# Autodesk Inventor assembly: EPS
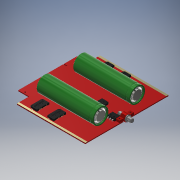
[picture p0: Inventor's stored thumbnail of the model, 180x180]
Saved by Autodesk Inventor 2018 (Build 220112000, 112)
## iProperties
Created: 2018-05-29
Part Number: EPS
Document SubType Name: Assembly
Designer: Bradley
Author: Bradley
## Documents named in this file (10)
- D:\Users\Bradley\Documents\CougsInSpace\CougSat1-Hardware\CougSat1-PowerBoard\CADModel\Native\EPS.iam
- D:\Users\Bradley\Documents\CougsInSpace\CougSat1-Hardware\CougSat1-PowerBoard\CADModel\Native\EPS_PCB.ipt
- D:\Users\Bradley\Documents\CougsInSpace\Resources\ComponentModels\Hardware\Pin_RBF.ipt
- D:\Users\Bradley\Documents\CougsInSpace\Resources\ComponentModels\Electronics\Switch_Micro-L.iam
- D:\Users\Bradley\Documents\CougsInSpace\Resources\ComponentModels\Electronics\Battery_18650.ipt
- D:\Users\Bradley\Documents\CougsInSpace\Resources\ComponentModels\Connectors\PicoLock--J-7.ipt
- D:\Users\Bradley\Documents\CougsInSpace\Resources\ComponentModels\Connectors\PicoLock--J-4.ipt
- D:\Users\Bradley\Documents\CougsInSpace\Resources\ComponentModels\Connectors\PicoLock--P-4.ipt
- D:\Users\Bradley\Documents\CougsInSpace\Resources\ComponentModels\Connectors\PicoLock--P-7.ipt
- D:\Users\Bradley\Documents\CougsInSpace\CougSat1-Hardware\CougSat1-PowerBoard\CADModel\Native\EPS_RBFPinHolder.ipt
## Components (16 placed, 9 different names)
1. EPS_PCB:1 — Mate:1, Angle:1, Flush:1, Flush:2, Mate:14, Mate:15, Mate:16, Mate:17, Mate:18, Flush:10, Flush:11, Flush:12, Flush:13, Flush:16, Mate:19, Insert:1, Insert:2
2. Pin_RBF:1 — Tangent:1, Insert:3
3. Switch_Micro-L:1 [sub-assembly] — Mate:1, Angle:1, Tangent:1, Mate:19
4. Battery_18650:1 — Flush:1, Flush:4, Symmetry:1
5. Battery_18650:2 — Flush:2, Flush:3, Symmetry:1
6. PicoLock--J-7:1 — Flush:6, Mate:6, Mate:7, Mate:14, Flush:10, Flush:14
7. PicoLock--J-4:1 — Flush:5, Mate:4, Mate:5, Mate:18
8. PicoLock--P-4:1 — Flush:5, Mate:4, Mate:5, Flush:16
9. PicoLock--P-7:1 — Flush:6, Mate:6, Mate:7
10. PicoLock--J-7:2 — Mate:15, Flush:11, Flush:15
11. PicoLock--P-7:2
12. PicoLock--J-7:3 — Mate:16, Flush:13, Flush:14
13. PicoLock--P-7:3
14. PicoLock--J-7:4 — Mate:17, Flush:12, Flush:15
15. PicoLock--P-7:4
16. EPS_RBFPinHolder:1 — Insert:1, Insert:2, Insert:3
## Relationships (39: Mate 17, Flush 16, Insert 3, Angle 1, Tangent 1, Symmetry 1)
- Mate:1: EPS_PCB:1 ↔ Switch_Micro-L:1
- Angle:1 (0 deg): EPS_PCB:1 ↔ Switch_Micro-L:1
- Tangent:1 (7.15 mm): Pin_RBF:1 ↔ Switch_Micro-L:1
- Flush:1 (-9 mm): EPS_PCB:1 ↔ Battery_18650:1
- Flush:2 (-9 mm): EPS_PCB:1 ↔ Battery_18650:2
- Flush:3 (-50 mm): Battery_18650:2
- Flush:4 (-50 mm): Battery_18650:1
- Symmetry:1: Battery_18650:1 ↔ Battery_18650:2
- Flush:5: PicoLock--J-4:1 ↔ PicoLock--P-4:1
- Mate:4: PicoLock--J-4:1 ↔ PicoLock--P-4:1
- Mate:5 (0.025 mm): PicoLock--J-4:1 ↔ PicoLock--P-4:1
- Flush:6: PicoLock--J-7:1 ↔ PicoLock--P-7:1
- Mate:6: PicoLock--J-7:1 ↔ PicoLock--P-7:1
- Mate:7 (0.025 mm): PicoLock--J-7:1 ↔ PicoLock--P-7:1
- [Flush]: PicoLock--J-7:2 ↔ PicoLock--P-7:2
- [Mate]: PicoLock--J-7:2 ↔ PicoLock--P-7:2
- [Mate] (0.025 mm): PicoLock--J-7:2 ↔ PicoLock--P-7:2
- [Flush]: PicoLock--J-7:3 ↔ PicoLock--P-7:3
- [Mate]: PicoLock--J-7:3 ↔ PicoLock--P-7:3
- [Mate] (0.025 mm): PicoLock--J-7:3 ↔ PicoLock--P-7:3
- [Flush]: PicoLock--J-7:4 ↔ PicoLock--P-7:4
- [Mate]: PicoLock--J-7:4 ↔ PicoLock--P-7:4
- [Mate] (0.025 mm): PicoLock--J-7:4 ↔ PicoLock--P-7:4
- Mate:14: EPS_PCB:1 ↔ PicoLock--J-7:1
- Mate:15: EPS_PCB:1 ↔ PicoLock--J-7:2
- Mate:16: EPS_PCB:1 ↔ PicoLock--J-7:3
- Mate:17: EPS_PCB:1 ↔ PicoLock--J-7:4
- Mate:18: EPS_PCB:1 ↔ PicoLock--J-4:1
- Flush:10 (-3 mm): EPS_PCB:1 ↔ PicoLock--J-7:1
- Flush:11 (-3 mm): EPS_PCB:1 ↔ PicoLock--J-7:2
- Flush:12 (-3 mm): EPS_PCB:1 ↔ PicoLock--J-7:4
- Flush:13 (-3 mm): EPS_PCB:1 ↔ PicoLock--J-7:3
- Flush:14: PicoLock--J-7:1 ↔ PicoLock--J-7:3
- Flush:15: PicoLock--J-7:2 ↔ PicoLock--J-7:4
- Flush:16 (-25 mm): EPS_PCB:1 ↔ PicoLock--P-4:1
- Mate:19 (-8.75 mm): EPS_PCB:1 ↔ Switch_Micro-L:1
- Insert:1: EPS_PCB:1 ↔ EPS_RBFPinHolder:1
- Insert:2: EPS_PCB:1 ↔ EPS_RBFPinHolder:1
- Insert:3: Pin_RBF:1 ↔ EPS_RBFPinHolder:1
## Named parameters: d15_d12 = 0 mm, d16_d13 = 0 mm, d17_d14 = 0.025 mm, d18_d12 = 0 mm, d19_d13 = 0 mm, d20_d14 = 0.025 mm, d21_d12 = 0 mm, d22_d13 = 0 mm, d23_d14 = 0.025 mm
